# Autodesk Inventor assembly: R-wing
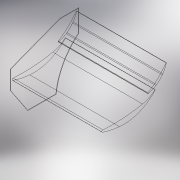
[picture p0: Inventor's stored thumbnail of the model, 180x180]
Saved by Autodesk Inventor 2018.2 (Build 222227000, 227)
## iProperties
Created: 2017-11-02
Part Number: R-wing
Material: 一般
Document SubType Name: Assembly
Designer: kuwano
Author: kuwano
## Documents named in this file (5)
- D:\kuwano\Documents\Inventor\KITformula\AeroCAD2018\CAD\Inventor\Aero Parts\R-wing\type6\R-wing.iam
- D:\kuwano\Documents\Inventor\KITformula\AeroCAD2018\CAD\Inventor\Aero Parts\R-wing\type6\parts\element_r_1.ipt
- D:\kuwano\Documents\Inventor\KITformula\AeroCAD2018\CAD\Inventor\Aero Parts\R-wing\type6\parts\end_plate.ipt
- D:\kuwano\Documents\Inventor\KITformula\AeroCAD2018\CAD\Inventor\Aero Parts\R-wing\type6\parts\end_plate_MIR.ipt
- D:\kuwano\Documents\Inventor\KITformula\AeroCAD2018\CAD\Inventor\Aero Parts\R-wing\type6\parts\cover_re.ipt
## Components (4 placed, 4 different names)
1. element_r_1:1 — フラッシュ:1, メイト:1, メイト:2
2. end_plate:1 — フラッシュ:3, フラッシュ:4, メイト:2, フラッシュ:6
3. end_plate_MIR:1 — フラッシュ:3, フラッシュ:4, メイト:1
4. cover_re:1 — フラッシュ:5
## Relationships (7: Flush 5, Mate 2)
- フラッシュ:1 [Flush]: element_r_1:1
- フラッシュ:3 [Flush]: end_plate:1 ↔ end_plate_MIR:1
- フラッシュ:4 [Flush]: end_plate:1 ↔ end_plate_MIR:1
- メイト:1 [Mate]: element_r_1:1 ↔ end_plate_MIR:1
- メイト:2 [Mate]: element_r_1:1 ↔ end_plate:1
- フラッシュ:5 [Flush]: cover_re:1
- フラッシュ:6 [Flush]: end_plate:1
